# Autodesk Inventor assembly: TR2 Arm
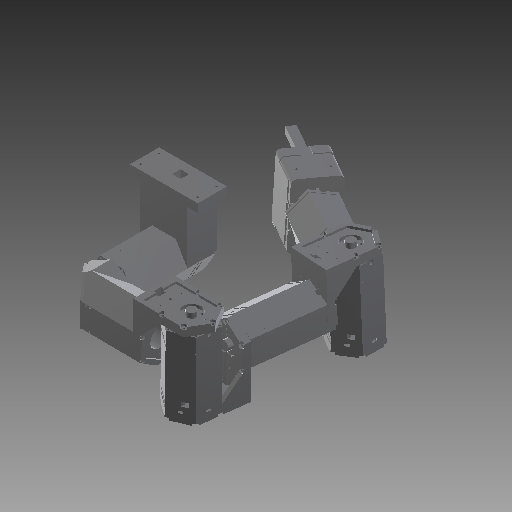
[picture p0: Inventor's stored thumbnail of the model, 512x512]
Saved by Autodesk Inventor 2017 (Build 210142000, 142)
## iProperties
Created: 2018-10-11
Part Number: TR2 Arm
Document SubType Name: Assembly
Designer: Zach
Author: Zach
## Documents named in this file (7)
- C:\Users\Dell\Documents\GitHub\tr2\Arm\Arm.iam
- C:\Users\Dell\Documents\GitHub\tr2\Arm\TARM01.ipt
- C:\Users\Dell\Documents\GitHub\tr2\Arm Actuator\Arm Actuator.iam
- C:\Users\Dell\Documents\GitHub\tr2\Arm\TARM02.ipt
- C:\Users\Dell\Documents\GitHub\tr2\Arm\TARM04.ipt
- C:\Users\Dell\Documents\GitHub\tr2\Arm\TARM08.ipt
- C:\Users\Dell\Documents\GitHub\tr2\Gripper\Gripper.iam
## Components (13 placed, 6 different names)
1. TARM01:1 — Mate:117, Mate:118, Mate:139
2. TARM02:1 — Mate:13, Mate:106, Mate:108, Mate:109, Mate:110, Mate:129, Mate:130, Mate:131
3. Arm Actuator:1 [sub-assembly] — Mate:13, Mate:106, Mate:117, Mate:118, Mate:139
4. Arm Actuator:2 [sub-assembly] — Mate:45, Mate:114, Mate:121, Mate:122, Mate:132, Mate:133
5. Arm Actuator:3 [sub-assembly] — Mate:48, Mate:113, Mate:134, Mate:135, Mate:136
6. Arm Actuator:4 [sub-assembly] — Mate:50, Mate:125, Mate:126, Mate:137, Mate:138
7. Arm Actuator:5 [sub-assembly] — Mate:53, Mate:112, Mate:127, Mate:128
8. TARM04:1 — Mate:45, Mate:48, Mate:113, Mate:114, Mate:121, Mate:122
9. TARM04:2 — Mate:50, Mate:53, Mate:112, Mate:125, Mate:126
10. TARM08:1 — Mate:108, Mate:109, Mate:110
11. Gripper:1 [sub-assembly] — Mate:127, Mate:128
12. TARM04:3 — Mate:129, Mate:130, Mate:131, Mate:132, Mate:133
13. TARM04:4 — Mate:134, Mate:135, Mate:136, Mate:137, Mate:138
## Relationships (31: Mate 31)
- Mate:13: TARM02:1 ↔ Arm Actuator:1
- Mate:45: Arm Actuator:2 ↔ TARM04:1
- Mate:48: Arm Actuator:3 ↔ TARM04:1
- Mate:50: Arm Actuator:4 ↔ TARM04:2
- Mate:53: Arm Actuator:5 ↔ TARM04:2
- Mate:106: TARM02:1 ↔ Arm Actuator:1
- Mate:108: TARM02:1 ↔ TARM08:1
- Mate:109: TARM02:1 ↔ TARM08:1
- Mate:110: TARM02:1 ↔ TARM08:1
- Mate:112: Arm Actuator:5 ↔ TARM04:2
- Mate:113: Arm Actuator:3 ↔ TARM04:1
- Mate:114: Arm Actuator:2 ↔ TARM04:1
- Mate:117: TARM01:1 ↔ Arm Actuator:1
- Mate:118: TARM01:1 ↔ Arm Actuator:1
- Mate:121: Arm Actuator:2 ↔ TARM04:1
- Mate:122: Arm Actuator:2 ↔ TARM04:1
- Mate:125: Arm Actuator:4 ↔ TARM04:2
- Mate:126: Arm Actuator:4 ↔ TARM04:2
- Mate:127: Arm Actuator:5 ↔ Gripper:1
- Mate:128: Arm Actuator:5 ↔ Gripper:1
- Mate:129: TARM02:1 ↔ TARM04:3
- Mate:130: TARM02:1 ↔ TARM04:3
- Mate:131: TARM02:1 ↔ TARM04:3
- Mate:132: Arm Actuator:2 ↔ TARM04:3
- Mate:133: Arm Actuator:2 ↔ TARM04:3
- Mate:134: Arm Actuator:3 ↔ TARM04:4
- Mate:135: Arm Actuator:3 ↔ TARM04:4
- Mate:136: Arm Actuator:3 ↔ TARM04:4
- Mate:137: Arm Actuator:4 ↔ TARM04:4
- Mate:138: Arm Actuator:4 ↔ TARM04:4
- Mate:139: TARM01:1 ↔ Arm Actuator:1
